# Autodesk Inventor assembly: striking
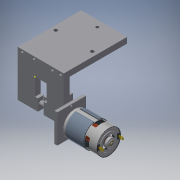
[picture p0: Inventor's stored thumbnail of the model, 180x180]
Saved by Autodesk Inventor 2019.4 (Build 234330000, 330)
## iProperties
Created: 2020-02-19
Part Number: striking
Document SubType Name: Assembly
Designer: Niran
Author: Niran
## Documents named in this file (10)
- C:\Users\Niran\Desktop\sketch_jan26a\Canon parts\striking.iam
- C:\Users\Niran\Desktop\sketch_jan26a\Canon parts\Part30.ipt
- C:\Users\Niran\Desktop\sketch_jan26a\Canon parts\Part33.ipt
- C:\Users\Niran\Desktop\sketch_jan26a\Canon parts\Part34.ipt
- C:\Users\Niran\Desktop\sketch_jan26a\Canon parts\Part35.ipt
- C:\Users\Niran\Desktop\sketch_jan26a\Canon parts\Part36.ipt
- C:\Users\Niran\Desktop\sketch_jan26a\Canon parts\DC Motor.ipt
- C:\Users\Niran\Desktop\sketch_jan26a\Canon parts\Part37.ipt
- C:\Users\Niran\Desktop\sketch_jan26a\Canon parts\Part38.ipt
- C:\Users\Niran\Desktop\sketch_jan26a\Canon parts\Part39.ipt
## Components (11 placed, 9 different names)
1. Part30:1 — Rigid:1
2. Part33:1 — Rigid:1, Rigid:2, Rigid:3
3. Part34:1 — Rigid:2, Rigid:5
4. Part34:2 — Rigid:3, Rigid:4
5. Part35:1 — Rigid:5
6. Part35:2 — Rigid:4, Rotational:1, Rigid:6
7. Part36:1 — Rotational:1, Rigid:7
8. DC Motor:1 — Rigid:6, Rigid:9
9. Part37:1 — Rigid:7, Rigid:8
10. Part38:1 — Rigid:8
11. Part39:1 — Rigid:9
## Relationships (10: WeldJoint 9, RevoluteJoint 1)
- Rigid:1 [WeldJoint]: Part30:1 ↔ Part33:1
- Rigid:2 [WeldJoint]: Part33:1 ↔ Part34:1
- Rigid:3 [WeldJoint]: Part33:1 ↔ Part34:2
- Rigid:4 [WeldJoint]: Part34:2 ↔ Part35:2
- Rigid:5 [WeldJoint]: Part34:1 ↔ Part35:1
- Rotational:1 [RevoluteJoint]: Part35:2 ↔ Part36:1
- Rigid:6 [WeldJoint] (4 mm): Part35:2 ↔ DC Motor:1
- Rigid:7 [WeldJoint]: Part36:1 ↔ Part37:1
- Rigid:8 [WeldJoint]: Part37:1 ↔ Part38:1
- Rigid:9 [WeldJoint]: DC Motor:1 ↔ Part39:1
